# Autodesk Inventor assembly: Drisk V0
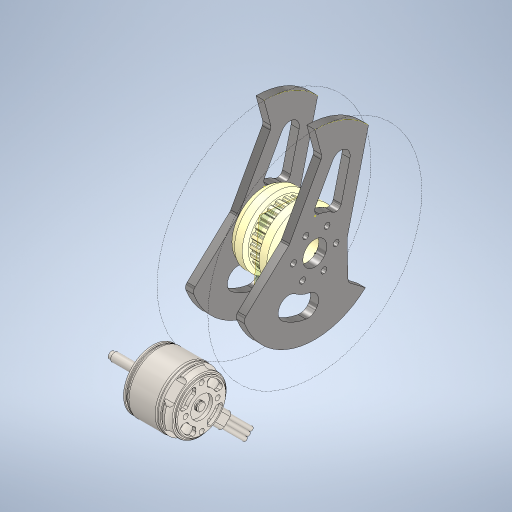
[picture p0: Inventor's stored thumbnail of the model, 512x512]
Saved by Autodesk Inventor 2023.4 (Build 274418000, 418)
## iProperties
Created: 2024-09-14
Part Number: Drisk V0
Document SubType Name: Assembly
Designer: Nathan Cai
Author: Nathan Cai
## Documents named in this file (4)
- E:\Documents\Inventor\Law - V2.1\Drisk V0\Drisk V0.iam
- E:\Documents\Inventor\Law - V2.1\Drisk V0\Flash_Hobby_D3536EVO v3\Flash_Hobby_D3536EVO v3.iam
- E:\Documents\Inventor\Law - V2.1\Drisk V0\Blade.ipt
- E:\Documents\Inventor\Law - V2.1\Drisk V0\XL Pulley Generator.ipt
## Components (4 placed, 3 different names)
1. Flash_Hobby_D3536EVO v3:1 [sub-assembly]
2. Blade:1 — Mate:1, Mate:2, Mate:3, Mate:6
3. Blade:2 — Mate:1, Mate:2, Mate:3, Mate:4, Mate:5
4. XL Pulley Generator:1 — Mate:4, Mate:5, Mate:6
## Relationships (6: Mate 6)
- Mate:1: Blade:1 ↔ Blade:2
- Mate:2: Blade:1 ↔ Blade:2
- Mate:3 (25.4 mm): Blade:1 ↔ Blade:2
- Mate:4: Blade:2 ↔ XL Pulley Generator:1
- Mate:5: Blade:2 ↔ XL Pulley Generator:1
- Mate:6: Blade:1 ↔ XL Pulley Generator:1
